# Autodesk Inventor assembly: StepperSystem
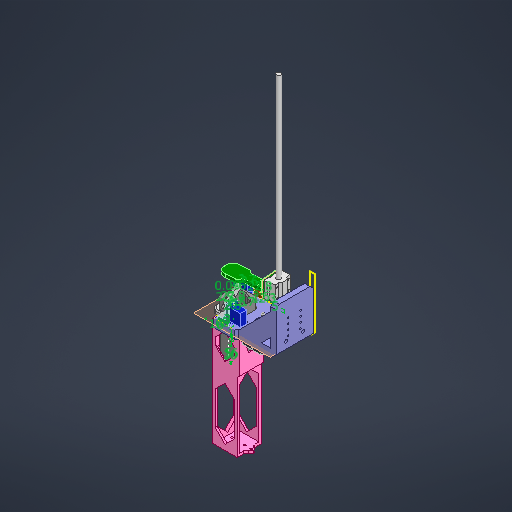
[picture p0: Inventor's stored thumbnail of the model, 512x512]
Saved by Autodesk Inventor 2025.1 (Build 291241000, 241)
## iProperties
Created: 2025-01-26
Part Number: StepperSystem
Document SubType Name: Assembly
Designer: 13156
Author: 13156
## Documents named in this file (21)
- C:\Users\jerem\Documents\GitHub\Perovskite-Automated-Synthesis-System\CAD\Pipette\StepperSystem.iam
- C:\Users\jerem\Documents\GitHub\Perovskite-Automated-Synthesis-System\CAD\Pipette\HolderWStepper.ipt
- C:\Users\jerem\Documents\GitHub\Perovskite-Automated-Synthesis-System\CAD\Non 3D Printed Parts\Linear Rails\8mm Linear Rod.ipt
- C:\Users\jerem\Documents\GitHub\Perovskite-Automated-Synthesis-System\CAD\Non 3D Printed Parts\Linear Rails\Linear Bearing 8mm Square.ipt
- C:\Users\jerem\Documents\GitHub\Perovskite-Automated-Synthesis-System\CAD\Pipette\Actuator.ipt
- C:\Users\jerem\Documents\GitHub\Perovskite-Automated-Synthesis-System\CAD\Pipette\PipetteStand.ipt
- C:\Users\jerem\Documents\GitHub\Perovskite-Automated-Synthesis-System\CAD\Non 3D Printed Parts\Motors and Servos\SG90 Servo.ipt
- C:\Users\jerem\Documents\GitHub\Perovskite-Automated-Synthesis-System\CAD\Pipette\GrabberArm.ipt
- C:\Users\jerem\Documents\GitHub\Perovskite-Automated-Synthesis-System\CAD\Pipette\SLEEVE.ipt
- C:\Users\jerem\Documents\GitHub\Perovskite-Automated-Synthesis-System\CAD\Non 3D Printed Parts\Leadscrew.ipt
- C:\Users\jerem\Documents\GitHub\Perovskite-Automated-Synthesis-System\CAD\Non 3D Printed Parts\Linear Rails\Linear Rod Holder SK8.ipt
- C:\Users\jerem\Documents\GitHub\Perovskite-Automated-Synthesis-System\CAD\Non 3D Printed Parts\Motors and Servos\NEMA17 Stepper Motor - 26 mm.ipt
- C:\Users\jerem\Documents\GitHub\Perovskite-Automated-Synthesis-System\CAD\Pipette\ServoHolder.ipt
- C:\Users\jerem\Documents\GitHub\Perovskite-Automated-Synthesis-System\CAD\Pipette\ServoHolder - short.ipt
- C:\Users\jerem\Documents\GitHub\Perovskite-Automated-Synthesis-System\CAD\Non 3D Printed Parts\Screws\M3x12.ipt
- C:\Users\jerem\Documents\GitHub\Perovskite-Automated-Synthesis-System\CAD\Non 3D Printed Parts\Screws\M2x8.ipt
- C:\Users\jerem\Documents\GitHub\Perovskite-Automated-Synthesis-System\CAD\Non 3D Printed Parts\Screws\M3x8.ipt
- C:\Users\jerem\Documents\GitHub\Perovskite-Automated-Synthesis-System\CAD\Pipette\HalfServoArm.ipt
- C:\Users\jerem\Documents\GitHub\Perovskite-Automated-Synthesis-System\CAD\Pipette\GrabberArmV2.ipt
- C:\Users\jerem\Documents\GitHub\Perovskite-Automated-Synthesis-System\CAD\Pipette\GrabberServoHolder.ipt
- C:\Users\jerem\Documents\GitHub\Perovskite-Automated-Synthesis-System\CAD\Pipette\EjectorArm.ipt
## Components (23 placed, 20 different names)
1. HolderWStepper:1 — Mate:9, Mate:13, Mate:14, Mate:15, Mate:16, Mate:25, Mate:26, Flush:4, Mate:46, Mate:47, Mate:50, Mate:51, Mate:54, Mate:95, Mate:96, Mate:97, Mate:100, Mate:101, Mate:102, Mate:111, Mate:112, Mate:114
2. 8mm Linear Rod:1 — Mate:21, Flush:4, Mate:48
3. Linear Bearing 8mm Square:1 — Mate:21, Mate:28, Mate:29, Mate:30, Mate:49
4. Actuator:1 — Mate:28, Mate:29, Mate:30, Mate:31, Mate:32, Mate:33, Mate:49
5. PipetteStand:1 — Mate:1, Mate:2, Mate:3, Mate:4, Mate:6, Mate:113
6. SG90 Servo:1 — Mate:98, Mate:99, Mate:115, Mate:116
7. GrabberArm:1 — Mate:77, Mate:78
8. Leadscrew:1 — Mate:31, Mate:32, Mate:33
9. Linear Rod Holder SK8:1 — Mate:13, Mate:14, Mate:15, Mate:16, Mate:48
10. SG90 Servo:3 — Mate:104, Mate:105, Mate:106, Mate:107, Angle:1
11. NEMA17 Stepper Motor - 26 mm:2 — Mate:9, Mate:25, Mate:26
12. SLEEVE:1 — Mate:4, Mate:6, Mate:46, Mate:47, Mate:54, Mate:77, Mate:78, Mate:92, Mate:95, Mate:103, Mate:113
13. ServoHolder:1 — Mate:50, Mate:51, Mate:63, Mate:64, Mate:65, Mate:66, Mate:69, Mate:70, Mate:104, Mate:105, Angle:1
14. ServoHolder - short:1 — Mate:96, Mate:97
15. M3x12:1 — Mate:63, Mate:64, Mate:70, Mate:111
16. M3x12:2 — Mate:65, Mate:66, Mate:69, Mate:112
17. M2x8:1
18. M3x8:1
19. HalfServoArm:1 — Mate:94, Mate:98, Mate:99
20. GrabberArmV2:1 — Mate:92, Mate:94, Mate:103
21. GrabberServoHolder:1 — Mate:100, Mate:101, Mate:102, Mate:114, Mate:115, Mate:116
22. EjectorArm:2 — Mate:108, Mate:109, Mate:110
23. HalfServoArm:2 — Mate:106, Mate:107, Mate:108, Mate:109, Mate:110
## Relationships (60: Mate 58, Flush 1, Angle 1)
- Mate:1: PipetteStand:1
- Mate:2: PipetteStand:1
- Mate:3: PipetteStand:1
- Mate:4: PipetteStand:1 ↔ SLEEVE:1
- Mate:6 (0.5 mm): PipetteStand:1 ↔ SLEEVE:1
- Mate:9: HolderWStepper:1 ↔ NEMA17 Stepper Motor - 26 mm:2
- Mate:13: HolderWStepper:1 ↔ Linear Rod Holder SK8:1
- Mate:14: HolderWStepper:1 ↔ Linear Rod Holder SK8:1
- Mate:15: HolderWStepper:1 ↔ Linear Rod Holder SK8:1
- Mate:16: HolderWStepper:1 ↔ Linear Rod Holder SK8:1
- Mate:21: 8mm Linear Rod:1 ↔ Linear Bearing 8mm Square:1
- Mate:25: HolderWStepper:1 ↔ NEMA17 Stepper Motor - 26 mm:2
- Mate:26: HolderWStepper:1 ↔ NEMA17 Stepper Motor - 26 mm:2
- Mate:28: Linear Bearing 8mm Square:1 ↔ Actuator:1
- Mate:29: Linear Bearing 8mm Square:1 ↔ Actuator:1
- Mate:30: Linear Bearing 8mm Square:1 ↔ Actuator:1
- Mate:31: Actuator:1 ↔ Leadscrew:1
- Mate:32: Actuator:1 ↔ Leadscrew:1
- Mate:33: Actuator:1 ↔ Leadscrew:1
- Flush:4: HolderWStepper:1 ↔ 8mm Linear Rod:1
- Mate:46: HolderWStepper:1 ↔ SLEEVE:1
- Mate:47: HolderWStepper:1 ↔ SLEEVE:1
- Mate:48: 8mm Linear Rod:1 ↔ Linear Rod Holder SK8:1
- Mate:49: Linear Bearing 8mm Square:1 ↔ Actuator:1
- Mate:50: HolderWStepper:1 ↔ ServoHolder:1
- Mate:51: HolderWStepper:1 ↔ ServoHolder:1
- Mate:54: HolderWStepper:1 ↔ SLEEVE:1
- Mate:63: ServoHolder:1 ↔ M3x12:1
- Mate:64: ServoHolder:1 ↔ M3x12:1
- Mate:65: ServoHolder:1 ↔ M3x12:2
- Mate:66: ServoHolder:1 ↔ M3x12:2
- Mate:69: ServoHolder:1 ↔ M3x12:2
- Mate:70: ServoHolder:1 ↔ M3x12:1
- Mate:77: GrabberArm:1 ↔ SLEEVE:1
- Mate:78: GrabberArm:1 ↔ SLEEVE:1
- Mate:92: SLEEVE:1 ↔ GrabberArmV2:1
- Mate:94: HalfServoArm:1 ↔ GrabberArmV2:1
- Mate:95: HolderWStepper:1 ↔ SLEEVE:1
- Mate:96: HolderWStepper:1 ↔ ServoHolder - short:1
- Mate:97: HolderWStepper:1 ↔ ServoHolder - short:1
- Mate:98: SG90 Servo:1 ↔ HalfServoArm:1
- Mate:99: SG90 Servo:1 ↔ HalfServoArm:1
- Mate:100: HolderWStepper:1 ↔ GrabberServoHolder:1
- Mate:101: HolderWStepper:1 ↔ GrabberServoHolder:1
- Mate:102: HolderWStepper:1 ↔ GrabberServoHolder:1
- Mate:103: SLEEVE:1 ↔ GrabberArmV2:1
- Mate:104: SG90 Servo:3 ↔ ServoHolder:1
- Mate:105: SG90 Servo:3 ↔ ServoHolder:1
- Mate:106: SG90 Servo:3 ↔ HalfServoArm:2
- Mate:107: SG90 Servo:3 ↔ HalfServoArm:2
- Mate:108: EjectorArm:2 ↔ HalfServoArm:2
- Mate:109: EjectorArm:2 ↔ HalfServoArm:2
- Mate:110: EjectorArm:2 ↔ HalfServoArm:2
- Mate:111: HolderWStepper:1 ↔ M3x12:1
- Mate:112: HolderWStepper:1 ↔ M3x12:2
- Angle:1 (0 deg): SG90 Servo:3 ↔ ServoHolder:1
- Mate:113: PipetteStand:1 ↔ SLEEVE:1
- Mate:114: HolderWStepper:1 ↔ GrabberServoHolder:1
- Mate:115: SG90 Servo:1 ↔ GrabberServoHolder:1
- Mate:116: SG90 Servo:1 ↔ GrabberServoHolder:1
